# Autodesk Inventor assembly: Frame
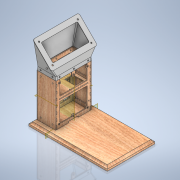
[picture p0: Inventor's stored thumbnail of the model, 180x180]
Saved by Autodesk Inventor 2020.2 (Build 242310000, 310)
## iProperties
Created: 2020-02-25
Part Number: Frame
Document SubType Name: Assembly
Designer: sdekr
Author: sdekr
## Documents named in this file (7)
- D:\Inventor\Project PAD\Frame.iam
- D:\Inventor\Project PAD\Base.ipt
- D:\Inventor\Project PAD\LCD mount to base.ipt
- D:\Inventor\Project PAD\Skeleton.ipt
- D:\Inventor\Project PAD\Back Plane.ipt
- D:\Inventor\Project PAD\Side Plane.ipt
- D:\Inventor\Project PAD\Front plane.ipt
## Components (7 placed, 6 different names)
1. Base:1 — Mate:1, Mate:2, Mate:3, Mate:16
2. Skeleton:1 — Mate:1, Mate:2, Mate:3, Mate:7, Mate:12, Mate:15, Mate:17, Mate:19, Mate:20
3. Back Plane:1 — Mate:7, Mate:14
4. Side Plane:1
5. Side Plane:2 — Mate:12, Mate:14
6. Front plane:1 — Mate:15, Mate:16
7. LCD mount to base:1 — Mate:17, Mate:19, Mate:20
## Relationships (11: Mate 11)
- Mate:1: Base:1 ↔ Skeleton:1
- Mate:2: Base:1 ↔ Skeleton:1
- Mate:3 (5 mm): Base:1 ↔ Skeleton:1
- Mate:7: Skeleton:1 ↔ Back Plane:1
- Mate:12: Skeleton:1 ↔ Side Plane:2
- Mate:14: Back Plane:1 ↔ Side Plane:2
- Mate:15: Skeleton:1 ↔ Front plane:1
- Mate:16: Base:1 ↔ Front plane:1
- Mate:17: Skeleton:1 ↔ LCD mount to base:1
- Mate:19: Skeleton:1 ↔ LCD mount to base:1
- Mate:20: Skeleton:1 ↔ LCD mount to base:1
